# Autodesk Inventor assembly: Atwoods2
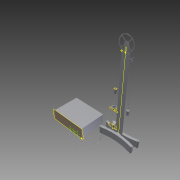
[picture p0: Inventor's stored thumbnail of the model, 180x180]
Saved by Autodesk Inventor 2012 SP2 (Build 160219200, 219)
## iProperties
Created: 2013-07-20
Part Number: Atwoods2
Document SubType Name: Assembly
Designer: 1
Author: 1
## Documents named in this file (15)
- D:\p3_metod1580library\figures\sources\M2-AlsoAtwoodsMachine\Atwoods2.iam
- D:\p3_metod1580library\figures\sources\M1-AtwoodsMachine\Atwoods-BaseBent.ipt
- D:\p3_metod1580library\figures\sources\M1-AtwoodsMachine\AdjLegStand.ipt
- D:\p3_metod1580library\figures\sources\M1-AtwoodsMachine\Ruler.ipt
- D:\p3_metod1580library\figures\sources\M2-AlsoAtwoodsMachine\Atwoods2-Wheel.ipt
- D:\p3_metod1580library\figures\sources\M2-AlsoAtwoodsMachine\WheelHolder.ipt
- D:\p3_metod1580library\figures\sources\M1-AtwoodsMachine\BallReciever.ipt
- D:\p3_metod1580library\figures\sources\M2-AlsoAtwoodsMachine\TriggerRing.ipt
- D:\p3_metod1580library\figures\sources\M1-AtwoodsMachine\AbstractBox.ipt
- D:\p3_metod1580library\figures\sources\M2-AlsoAtwoodsMachine\ThreadBreak.ipt
- D:\p3_metod1580library\figures\sources\M2-AlsoAtwoodsMachine\M2Thread.ipt
- D:\p3_metod1580library\figures\sources\M2-AlsoAtwoodsMachine\AtwoodsMass.ipt
- D:\p3_metod1580library\figures\sources\M2-AlsoAtwoodsMachine\Wire1.ipt
- D:\p3_metod1580library\figures\sources\M2-AlsoAtwoodsMachine\Wire2.ipt
- D:\p3_metod1580library\figures\sources\M2-AlsoAtwoodsMachine\Wire3.ipt
## Components (19 placed, 14 different names)
1. AdjLegStand:1 — Insert:4, Flush:14
2. AdjLegStand:2 — Insert:1
3. AdjLegStand:3 — Insert:3
4. AdjLegStand:4 — Insert:2
5. Ruler:1 — Mate:4, Mate:6, Mate:7, Angle:2, Flush:4, Mate:9, Mate:10, Mate:11, Angle:5, Mate:12, Angle:7, Mate:13, Flush:7
6. Atwoods2-Wheel:1 — Flush:3
7. WheelHolder:1 — Flush:4
8. Atwoods-BaseBent:1 — Mate:8, Flush:5, Flush:6, Mate:9, Mate:10, Mate:11, Insert:3, Insert:4
9. Atwoods-BaseBent:2 — Mate:8, Flush:5, Flush:6, Insert:1, Insert:2
10. BallReciever:1 — Mate:13, Flush:7
11. TriggerRing:1 — Flush:8
12. AbstractBox:1 — Flush:14, Flush:18, Flush:19, Flush:20
13. ThreadBreak:1 — Flush:15, Flush:21
14. M2Thread:1 — Flush:16, Flush:17, Insert:5
15. AtwoodsMass:1 — Flush:17
16. AtwoodsMass:2 — Insert:5
17. Wire1:1 — Flush:18, Flush:19
18. Wire2:1 — Flush:20
19. Wire3:1 — Flush:21
## Relationships (32: Flush 14, Mate 9, Insert 5, Angle 4)
- Mate:4: Ruler:1
- Mate:6: Ruler:1
- Mate:7: Ruler:1
- Angle:2 (0 deg): Ruler:1
- Flush:3: Atwoods2-Wheel:1
- Flush:4: Ruler:1 ↔ WheelHolder:1
- Mate:8: Atwoods-BaseBent:1 ↔ Atwoods-BaseBent:2
- Flush:5: Atwoods-BaseBent:1 ↔ Atwoods-BaseBent:2
- Flush:6: Atwoods-BaseBent:1 ↔ Atwoods-BaseBent:2
- Mate:9: Ruler:1 ↔ Atwoods-BaseBent:1
- Mate:10: Ruler:1 ↔ Atwoods-BaseBent:1
- Mate:11: Ruler:1 ↔ Atwoods-BaseBent:1
- Insert:1: AdjLegStand:2 ↔ Atwoods-BaseBent:2
- Insert:2: AdjLegStand:4 ↔ Atwoods-BaseBent:2
- Insert:3: AdjLegStand:3 ↔ Atwoods-BaseBent:1
- Insert:4: AdjLegStand:1 ↔ Atwoods-BaseBent:1
- Angle:5 (0 deg): Ruler:1
- Mate:12: Ruler:1
- Angle:6 (0 deg)
- Angle:7 (0 deg): Ruler:1
- Mate:13 (-21 mm): Ruler:1 ↔ BallReciever:1
- Flush:7: Ruler:1 ↔ BallReciever:1
- Flush:8: TriggerRing:1
- Flush:14: AdjLegStand:1 ↔ AbstractBox:1
- Flush:15: ThreadBreak:1
- Flush:16: M2Thread:1
- Flush:17: M2Thread:1 ↔ AtwoodsMass:1
- Insert:5: M2Thread:1 ↔ AtwoodsMass:2
- Flush:18: AbstractBox:1 ↔ Wire1:1
- Flush:19: AbstractBox:1 ↔ Wire1:1
- Flush:20: AbstractBox:1 ↔ Wire2:1
- Flush:21: ThreadBreak:1 ↔ Wire3:1
